# Autodesk Inventor assembly: Rat_Scanner_120_Ass
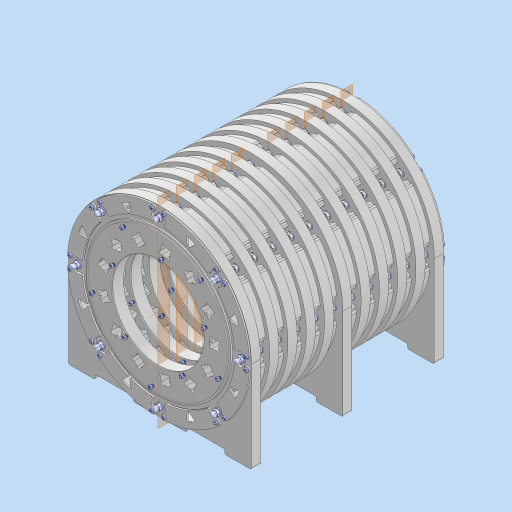
[picture p0: Inventor's stored thumbnail of the model, 512x512]
Saved by Autodesk Inventor 2024.2 (Build 282272000, 272)
## iProperties
Created: 2025-04-30
Part Number: Rat_Scanner_120_Ass
Document SubType Name: Assembly
Designer: 23661194
Author: 23661194
## Documents named in this file (14)
- C:\Users\23661194\OneDrive - Stellenbosch University\Master 2025 - Rat Scanner (120mm)\Rat_Scanner_120_V1\Rat_Scanner_120_Ass.iam
- C:\Users\23661194\OneDrive - Stellenbosch University\Master 2025 - Rat Scanner (120mm)\Rat_Scanner_120_V1\Ring_842_Sub.iam
- C:\Users\23661194\OneDrive - Stellenbosch University\Master 2025 - Rat Scanner (120mm)\Rat_Scanner_120_V1\Ring_945_Sub.iam
- C:\Users\23661194\OneDrive - Stellenbosch University\Master 2025 - Rat Scanner (120mm)\Rat_Scanner_120_V1\Ring_1050_Sub.iam
- C:\Users\23661194\OneDrive - Stellenbosch University\Master 2025 - Rat Scanner (120mm)\Rat_Scanner_120_V1\Ring_0_Sub.iam
- C:\Users\23661194\OneDrive - Stellenbosch University\Master 2025 - Rat Scanner (120mm)\Rat_Scanner_120_V1\Ring_1_Sub.iam
- C:\Users\23661194\OneDrive - Stellenbosch University\Master 2025 - Rat Scanner (120mm)\Rat_Scanner_120_V1\Ring_10_Sub.iam
- C:\Users\23661194\OneDrive - Stellenbosch University\Master 2025 - Rat Scanner (120mm)\Rat_Scanner_120_V1\Brass_Rod_M4.ipt
- C:\Users\23661194\OneDrive - Stellenbosch University\Master 2025 - Rat Scanner (120mm)\Rat_Scanner_120_V1\M4_Nylon_Washer.ipt
- C:\Users\23661194\OneDrive - Stellenbosch University\Master 2025 - Rat Scanner (120mm)\Rat_Scanner_120_V1\M4x3.2mm Hex Nut.ipt
- C:\Users\23661194\OneDrive - Stellenbosch University\Master 2025 - Rat Scanner (120mm)\Rat_Scanner_120_V1\M4 Dome Nut.ipt
- C:\Users\23661194\OneDrive - Stellenbosch University\Master 2025 - Rat Scanner (120mm)\Rat_Scanner_120_V1\Shim_Tray.ipt
- C:\Users\23661194\OneDrive - Stellenbosch University\Master 2025 - Rat Scanner (120mm)\Rat_Scanner_120_V1\Ring_10_Back_Sub.iam
- C:\Users\23661194\OneDrive - Stellenbosch University\Master 2025 - Rat Scanner (120mm)\Rat_Scanner_120_V1\M3x8.ipt
## Components (419 placed, 13 different names)
1. Ring_842_Sub:1 [sub-assembly] — Mate:1, Flush:1, Mate:2, Mate:3, Flush:2, Mate:4, Mate:5, Flush:3, Mate:7, Flush:4, Mate:10, Flush:5, Mate:12, Flush:6, Mate:15, Flush:7, Mate:17, Flush:8, Flush:10, Mate:51
2. Ring_945_Sub:1 [sub-assembly] — Mate:1, Flush:1, Mate:2, Mate:6, Mate:21, Flush:11
3. Ring_945_Sub:2 [sub-assembly] — Mate:3, Flush:2, Mate:4, Mate:8, Mate:39
4. Ring_1050_Sub:1 [sub-assembly] — Mate:5, Flush:3, Mate:6, Mate:9
5. Ring_1050_Sub:2 [sub-assembly] — Mate:7, Flush:4, Mate:8, Mate:11
6. Ring_0_Sub:1 [sub-assembly] — Mate:11, Mate:12, Flush:6, Mate:14
7. Ring_0_Sub:2 [sub-assembly] — Mate:9, Mate:10, Flush:5, Mate:16
8. Ring_1_Sub:1 [sub-assembly] — Mate:14, Mate:15, Flush:7, Mate:20
9. Ring_1_Sub:2 [sub-assembly] — Mate:16, Mate:17, Flush:8, Mate:38
10. Ring_10_Sub:2 [sub-assembly] — Mate:20, Mate:21, Flush:10, Mate:35, Mate:36, Mate:37, Mate:47, Mate:49, Mate:52
11. Ring_10_Back_Sub:1 [sub-assembly] — Mate:38, Mate:39, Flush:11, Mate:40, Mate:41, Mate:42, Mate:43, Mate:45, Flush:12, Mate:54
12. Shim_Tray:2 — Mate:40, Mate:41, Mate:42, Mate:44, Mate:46
13. M3x8:2 — Mate:45, Mate:46
14. M3x8:1 — Mate:43, Mate:44
15. Shim_Tray:3
16. M3x8:3
17. M3x8:4
18. Shim_Tray:4
19. M3x8:5
20. M3x8:6
21. Shim_Tray:5
22. M3x8:7
23. M3x8:8
24. Shim_Tray:6
25. M3x8:9
26. M3x8:10
27. Shim_Tray:7
28. M3x8:11
29. M3x8:12
30. Shim_Tray:8
31. M3x8:13
32. M3x8:14
33. Shim_Tray:9
34. M3x8:15
35. M3x8:16
36. Shim_Tray:1 — Mate:35, Mate:36, Mate:37, Mate:48, Mate:50
37. M3x8:17 — Mate:47, Mate:48
38. M3x8:18 — Mate:49, Mate:50
39. Shim_Tray:10
40. M3x8:19
41. M3x8:20
42. Shim_Tray:11
43. M3x8:21
44. M3x8:22
45. Shim_Tray:12
46. M3x8:23
47. M3x8:24
48. Shim_Tray:13
49. M3x8:25
50. M3x8:26
51. Shim_Tray:14
52. M3x8:27
53. M3x8:28
54. Shim_Tray:15
55. M3x8:29
56. M3x8:30
57. Shim_Tray:16
58. M3x8:31
59. M3x8:32
60. Brass_Rod_M4:1 — Mate:51, Flush:12
61. Brass_Rod_M4:2 — Mate:53, Mate:55, Mate:56, Mate:57, Mate:60, Mate:62
62. Brass_Rod_M4:3
63. Brass_Rod_M4:4
64. Brass_Rod_M4:5
65. Brass_Rod_M4:6
66. Brass_Rod_M4:7
67. Brass_Rod_M4:8
68. M4 Dome Nut:1 — Mate:56, Mate:59
69. M4 Dome Nut:2 — Mate:57, Mate:58
70. M4 Dome Nut:3
71. M4 Dome Nut:4
72. M4 Dome Nut:5
73. M4 Dome Nut:6
74. M4 Dome Nut:7
75. M4 Dome Nut:8
76. M4 Dome Nut:9
77. M4 Dome Nut:10
78. M4 Dome Nut:11
79. M4 Dome Nut:12
80. M4 Dome Nut:13
81. M4 Dome Nut:14
82. M4 Dome Nut:15
83. M4 Dome Nut:16
84. M4_Nylon_Washer:2 — Mate:52, Mate:53, Mate:59
85. M4_Nylon_Washer:3
86. M4_Nylon_Washer:4
87. M4_Nylon_Washer:5
88. M4_Nylon_Washer:6
89. M4_Nylon_Washer:7
90. M4_Nylon_Washer:8
91. M4_Nylon_Washer:9
92. M4_Nylon_Washer:10 — Mate:63
93. M4_Nylon_Washer:11
94. M4_Nylon_Washer:12
95. M4_Nylon_Washer:13
96. M4_Nylon_Washer:14
97. M4_Nylon_Washer:15
98. M4_Nylon_Washer:16
99. M4_Nylon_Washer:17
100. M4_Nylon_Washer:18
101. M4_Nylon_Washer:19
102. M4_Nylon_Washer:20
103. M4_Nylon_Washer:21
104. M4_Nylon_Washer:22
105. M4_Nylon_Washer:23
106. M4_Nylon_Washer:24
107. M4_Nylon_Washer:25
108. M4_Nylon_Washer:26
109. M4_Nylon_Washer:27
110. M4_Nylon_Washer:28
111. M4_Nylon_Washer:29
112. M4_Nylon_Washer:30
113. M4_Nylon_Washer:31
114. M4_Nylon_Washer:32
115. M4_Nylon_Washer:33
116. M4_Nylon_Washer:34
117. M4_Nylon_Washer:35
118. M4_Nylon_Washer:36
119. M4_Nylon_Washer:37
120. M4_Nylon_Washer:38
121. M4_Nylon_Washer:39
122. M4_Nylon_Washer:40
123. M4_Nylon_Washer:41
124. M4_Nylon_Washer:42
125. M4_Nylon_Washer:43
126. M4_Nylon_Washer:44
127. M4_Nylon_Washer:45
128. M4_Nylon_Washer:46
129. M4_Nylon_Washer:47
130. M4_Nylon_Washer:48
131. M4_Nylon_Washer:49
132. M4_Nylon_Washer:50
133. M4_Nylon_Washer:51
134. M4_Nylon_Washer:52
135. M4_Nylon_Washer:53
136. M4_Nylon_Washer:54
137. M4_Nylon_Washer:55
138. M4_Nylon_Washer:56
139. M4_Nylon_Washer:57
140. M4_Nylon_Washer:58
141. M4_Nylon_Washer:59
142. M4_Nylon_Washer:60
143. M4_Nylon_Washer:61
144. M4_Nylon_Washer:62
145. M4_Nylon_Washer:63
146. M4_Nylon_Washer:64
147. M4_Nylon_Washer:65
148. M4_Nylon_Washer:66
149. M4_Nylon_Washer:67
150. M4_Nylon_Washer:68
151. M4_Nylon_Washer:69
152. M4_Nylon_Washer:70
153. M4_Nylon_Washer:71
154. M4_Nylon_Washer:72
155. M4_Nylon_Washer:73
156. M4_Nylon_Washer:74
157. M4_Nylon_Washer:75
158. M4_Nylon_Washer:76
159. M4_Nylon_Washer:77
160. M4_Nylon_Washer:78
161. M4_Nylon_Washer:79
162. M4_Nylon_Washer:80
163. M4_Nylon_Washer:81
164. M4_Nylon_Washer:82
165. M4_Nylon_Washer:83
166. M4_Nylon_Washer:84
167. M4_Nylon_Washer:85
168. M4_Nylon_Washer:86
169. M4_Nylon_Washer:87
170. M4_Nylon_Washer:88
171. M4_Nylon_Washer:89
172. M4_Nylon_Washer:90 — Mate:54, Mate:55, Mate:58
173. M4_Nylon_Washer:91
174. M4_Nylon_Washer:92
175. M4_Nylon_Washer:93
176. M4_Nylon_Washer:94
177. M4_Nylon_Washer:95
178. M4_Nylon_Washer:96
179. M4_Nylon_Washer:97
180. M4_Nylon_Washer:98
181. M4_Nylon_Washer:99
182. M4_Nylon_Washer:100
183. M4_Nylon_Washer:101
184. M4_Nylon_Washer:102
185. M4_Nylon_Washer:103
186. M4_Nylon_Washer:104
187. M4_Nylon_Washer:105
188. M4_Nylon_Washer:106
189. M4_Nylon_Washer:107
190. M4_Nylon_Washer:108
191. M4_Nylon_Washer:109
192. M4_Nylon_Washer:110
193. M4_Nylon_Washer:111
194. M4_Nylon_Washer:112
195. M4_Nylon_Washer:113
196. M4_Nylon_Washer:114
197. M4_Nylon_Washer:115
198. M4_Nylon_Washer:116
199. M4_Nylon_Washer:117
200. M4_Nylon_Washer:118
201. M4_Nylon_Washer:119
202. M4_Nylon_Washer:120
203. M4_Nylon_Washer:121
204. M4_Nylon_Washer:122
205. M4_Nylon_Washer:123
206. M4_Nylon_Washer:124
207. M4_Nylon_Washer:125
208. M4_Nylon_Washer:126
209. M4_Nylon_Washer:127
210. M4_Nylon_Washer:128
211. M4_Nylon_Washer:129
212. M4_Nylon_Washer:130
213. M4_Nylon_Washer:131
214. M4_Nylon_Washer:132
215. M4_Nylon_Washer:133
216. M4_Nylon_Washer:134
217. M4_Nylon_Washer:135
218. M4_Nylon_Washer:136
219. M4_Nylon_Washer:137
220. M4_Nylon_Washer:138
221. M4_Nylon_Washer:139
222. M4_Nylon_Washer:140
223. M4_Nylon_Washer:141
224. M4_Nylon_Washer:142
225. M4_Nylon_Washer:143
226. M4_Nylon_Washer:144
227. M4_Nylon_Washer:145
228. M4_Nylon_Washer:146
229. M4_Nylon_Washer:147
230. M4_Nylon_Washer:148
231. M4_Nylon_Washer:149
232. M4_Nylon_Washer:150
233. M4_Nylon_Washer:151
234. M4_Nylon_Washer:152
235. M4_Nylon_Washer:153
236. M4_Nylon_Washer:154
237. M4_Nylon_Washer:155
238. M4_Nylon_Washer:156
239. M4_Nylon_Washer:157
240. M4_Nylon_Washer:158
241. M4_Nylon_Washer:159
242. M4_Nylon_Washer:160
243. M4_Nylon_Washer:161
244. M4_Nylon_Washer:162
245. M4_Nylon_Washer:163
246. M4_Nylon_Washer:164
247. M4_Nylon_Washer:165
248. M4_Nylon_Washer:166
249. M4_Nylon_Washer:167
250. M4_Nylon_Washer:168
251. M4_Nylon_Washer:169
252. M4_Nylon_Washer:170 — Mate:61
253. M4_Nylon_Washer:171
254. M4_Nylon_Washer:172
255. M4_Nylon_Washer:173
256. M4_Nylon_Washer:174
257. M4_Nylon_Washer:175
258. M4_Nylon_Washer:176
259. M4_Nylon_Washer:177
260. M4x3.2mm Hex Nut:2 — Mate:62, Mate:63
261. M4x3.2mm Hex Nut:1 — Mate:60, Mate:61
262. M4x3.2mm Hex Nut:3
263. M4x3.2mm Hex Nut:4
264. M4x3.2mm Hex Nut:5
265. M4x3.2mm Hex Nut:6
266. M4x3.2mm Hex Nut:7
267. M4x3.2mm Hex Nut:8
268. M4x3.2mm Hex Nut:9
269. M4x3.2mm Hex Nut:10
270. M4x3.2mm Hex Nut:11
271. M4x3.2mm Hex Nut:12
272. M4x3.2mm Hex Nut:13
273. M4x3.2mm Hex Nut:14
274. M4x3.2mm Hex Nut:15
275. M4x3.2mm Hex Nut:16
276. M4x3.2mm Hex Nut:17
277. M4x3.2mm Hex Nut:18
278. M4x3.2mm Hex Nut:19
279. M4x3.2mm Hex Nut:20
280. M4x3.2mm Hex Nut:21
281. M4x3.2mm Hex Nut:22
282. M4x3.2mm Hex Nut:23
283. M4x3.2mm Hex Nut:24
284. M4x3.2mm Hex Nut:25
285. M4x3.2mm Hex Nut:26
286. M4x3.2mm Hex Nut:27
287. M4x3.2mm Hex Nut:28
288. M4x3.2mm Hex Nut:29
289. M4x3.2mm Hex Nut:30
290. M4x3.2mm Hex Nut:31
291. M4x3.2mm Hex Nut:32
292. M4x3.2mm Hex Nut:33
293. M4x3.2mm Hex Nut:34
294. M4x3.2mm Hex Nut:35
295. M4x3.2mm Hex Nut:36
296. M4x3.2mm Hex Nut:37
297. M4x3.2mm Hex Nut:38
298. M4x3.2mm Hex Nut:39
299. M4x3.2mm Hex Nut:40
300. M4x3.2mm Hex Nut:41
301. M4x3.2mm Hex Nut:42
302. M4x3.2mm Hex Nut:43
303. M4x3.2mm Hex Nut:44
304. M4x3.2mm Hex Nut:45
305. M4x3.2mm Hex Nut:46
306. M4x3.2mm Hex Nut:47
307. M4x3.2mm Hex Nut:48
308. M4x3.2mm Hex Nut:49
309. M4x3.2mm Hex Nut:50
310. M4x3.2mm Hex Nut:51
311. M4x3.2mm Hex Nut:52
312. M4x3.2mm Hex Nut:53
313. M4x3.2mm Hex Nut:54
314. M4x3.2mm Hex Nut:55
315. M4x3.2mm Hex Nut:56
316. M4x3.2mm Hex Nut:57
317. M4x3.2mm Hex Nut:58
318. M4x3.2mm Hex Nut:59
319. M4x3.2mm Hex Nut:60
320. M4x3.2mm Hex Nut:61
321. M4x3.2mm Hex Nut:62
322. M4x3.2mm Hex Nut:63
323. M4x3.2mm Hex Nut:64
324. M4x3.2mm Hex Nut:65
325. M4x3.2mm Hex Nut:66
326. M4x3.2mm Hex Nut:67
327. M4x3.2mm Hex Nut:68
328. M4x3.2mm Hex Nut:69
329. M4x3.2mm Hex Nut:70
330. M4x3.2mm Hex Nut:71
331. M4x3.2mm Hex Nut:72
332. M4x3.2mm Hex Nut:73
333. M4x3.2mm Hex Nut:74
334. M4x3.2mm Hex Nut:75
335. M4x3.2mm Hex Nut:76
336. M4x3.2mm Hex Nut:77
337. M4x3.2mm Hex Nut:78
338. M4x3.2mm Hex Nut:79
339. M4x3.2mm Hex Nut:80
340. M4x3.2mm Hex Nut:81
341. M4x3.2mm Hex Nut:82
342. M4x3.2mm Hex Nut:83
343. M4x3.2mm Hex Nut:84
344. M4x3.2mm Hex Nut:85
345. M4x3.2mm Hex Nut:86
346. M4x3.2mm Hex Nut:87
347. M4x3.2mm Hex Nut:88
348. M4x3.2mm Hex Nut:89
349. M4x3.2mm Hex Nut:90
350. M4x3.2mm Hex Nut:91
351. M4x3.2mm Hex Nut:92
352. M4x3.2mm Hex Nut:93
353. M4x3.2mm Hex Nut:94
354. M4x3.2mm Hex Nut:95
355. M4x3.2mm Hex Nut:96
356. M4x3.2mm Hex Nut:97
357. M4x3.2mm Hex Nut:98
358. M4x3.2mm Hex Nut:99
359. M4x3.2mm Hex Nut:100
360. M4x3.2mm Hex Nut:101
361. M4x3.2mm Hex Nut:102
362. M4x3.2mm Hex Nut:103
363. M4x3.2mm Hex Nut:104
364. M4x3.2mm Hex Nut:105
365. M4x3.2mm Hex Nut:106
366. M4x3.2mm Hex Nut:107
367. M4x3.2mm Hex Nut:108
368. M4x3.2mm Hex Nut:109
369. M4x3.2mm Hex Nut:110
370. M4x3.2mm Hex Nut:111
371. M4x3.2mm Hex Nut:112
372. M4x3.2mm Hex Nut:113
373. M4x3.2mm Hex Nut:114
374. M4x3.2mm Hex Nut:115
375. M4x3.2mm Hex Nut:116
376. M4x3.2mm Hex Nut:117
377. M4x3.2mm Hex Nut:118
378. M4x3.2mm Hex Nut:119
379. M4x3.2mm Hex Nut:120
380. M4x3.2mm Hex Nut:121
381. M4x3.2mm Hex Nut:122
382. M4x3.2mm Hex Nut:123
383. M4x3.2mm Hex Nut:124
384. M4x3.2mm Hex Nut:125
385. M4x3.2mm Hex Nut:126
386. M4x3.2mm Hex Nut:127
387. M4x3.2mm Hex Nut:128
388. M4x3.2mm Hex Nut:129
389. M4x3.2mm Hex Nut:130
390. M4x3.2mm Hex Nut:131
391. M4x3.2mm Hex Nut:132
392. M4x3.2mm Hex Nut:133
393. M4x3.2mm Hex Nut:134
394. M4x3.2mm Hex Nut:135
395. M4x3.2mm Hex Nut:136
396. M4x3.2mm Hex Nut:137
397. M4x3.2mm Hex Nut:138
398. M4x3.2mm Hex Nut:139
399. M4x3.2mm Hex Nut:140
400. M4x3.2mm Hex Nut:141
401. M4x3.2mm Hex Nut:142
402. M4x3.2mm Hex Nut:143
403. M4x3.2mm Hex Nut:144
404. M4x3.2mm Hex Nut:145
405. M4x3.2mm Hex Nut:146
406. M4x3.2mm Hex Nut:147
407. M4x3.2mm Hex Nut:148
408. M4x3.2mm Hex Nut:149
409. M4x3.2mm Hex Nut:150
410. M4x3.2mm Hex Nut:151
411. M4x3.2mm Hex Nut:152
412. M4x3.2mm Hex Nut:153
413. M4x3.2mm Hex Nut:154
414. M4x3.2mm Hex Nut:155
415. M4x3.2mm Hex Nut:156
416. M4x3.2mm Hex Nut:157
417. M4x3.2mm Hex Nut:158
418. M4x3.2mm Hex Nut:159
419. M4x3.2mm Hex Nut:160
## Component patterns: (8 elements, first: Shim_Tray:2 + M3x8:2 + M3x8:1), (8 elements, first: Shim_Tray:1 + M3x8:17 + M3x8:18), (8 elements, first: Brass_Rod_M4:1), (11 elements), (11 elements), (8 elements, first: M4 Dome Nut:1 + M4 Dome Nut:2), (10 elements), (8 elements, first: M4_Nylon_Washer:2), Component Pattern 15:2 (8 elements), Component Pattern 15:3 (8 elements), Component Pattern 15:4 (8 elements), Component Pattern 15:5 (8 elements), Component Pattern 15:6 (8 elements), Component Pattern 15:7 (8 elements), Component Pattern 15:8 (8 elements), Component Pattern 15:9 (8 elements), Component Pattern 15:10 (8 elements), Component Pattern 15:11 (8 elements), (8 elements, first: M4_Nylon_Washer:90), Component Pattern 17:2 (8 elements), Component Pattern 17:3 (8 elements), Component Pattern 17:4 (8 elements), Component Pattern 17:5 (8 elements), Component Pattern 17:6 (8 elements), Component Pattern 17:7 (8 elements), Component Pattern 17:8 (8 elements), Component Pattern 17:9 (8 elements), Component Pattern 17:10 (8 elements), Component Pattern 17:11 (8 elements), (8 elements, first: M4x3.2mm Hex Nut:2 + M4x3.2mm Hex Nut:1), Component Pattern 20:2 (8 elements), Component Pattern 20:3 (8 elements), Component Pattern 20:4 (8 elements), Component Pattern 20:5 (8 elements), Component Pattern 20:6 (8 elements), Component Pattern 20:7 (8 elements), Component Pattern 20:8 (8 elements), Component Pattern 20:9 (8 elements), Component Pattern 20:10 (8 elements)
## Relationships (58: Mate 47, Flush 11)
- Mate:1: Ring_842_Sub:1 ↔ Ring_945_Sub:1
- Flush:1: Ring_842_Sub:1 ↔ Ring_945_Sub:1
- Mate:2 (12 mm): Ring_842_Sub:1 ↔ Ring_945_Sub:1
- Mate:3: Ring_842_Sub:1 ↔ Ring_945_Sub:2
- Flush:2: Ring_842_Sub:1 ↔ Ring_945_Sub:2
- Mate:4 (12 mm): Ring_842_Sub:1 ↔ Ring_945_Sub:2
- Mate:5: Ring_842_Sub:1 ↔ Ring_1050_Sub:1
- Flush:3: Ring_842_Sub:1 ↔ Ring_1050_Sub:1
- Mate:6 (12 mm): Ring_945_Sub:1 ↔ Ring_1050_Sub:1
- Mate:7: Ring_842_Sub:1 ↔ Ring_1050_Sub:2
- Flush:4: Ring_842_Sub:1 ↔ Ring_1050_Sub:2
- Mate:8 (12 mm): Ring_945_Sub:2 ↔ Ring_1050_Sub:2
- Mate:9 (12 mm): Ring_1050_Sub:1 ↔ Ring_0_Sub:2
- Mate:10: Ring_842_Sub:1 ↔ Ring_0_Sub:2
- Flush:5: Ring_842_Sub:1 ↔ Ring_0_Sub:2
- Mate:11 (12 mm): Ring_1050_Sub:2 ↔ Ring_0_Sub:1
- Mate:12: Ring_842_Sub:1 ↔ Ring_0_Sub:1
- Flush:6: Ring_842_Sub:1 ↔ Ring_0_Sub:1
- Mate:14 (12 mm): Ring_0_Sub:1 ↔ Ring_1_Sub:1
- Mate:15: Ring_842_Sub:1 ↔ Ring_1_Sub:1
- Flush:7: Ring_842_Sub:1 ↔ Ring_1_Sub:1
- Mate:16 (12 mm): Ring_0_Sub:2 ↔ Ring_1_Sub:2
- Mate:17: Ring_842_Sub:1 ↔ Ring_1_Sub:2
- Flush:8: Ring_842_Sub:1 ↔ Ring_1_Sub:2
- Mate:20 (12 mm): Ring_1_Sub:1 ↔ Ring_10_Sub:2
- Mate:21: Ring_945_Sub:1 ↔ Ring_10_Sub:2
- Flush:10: Ring_842_Sub:1 ↔ Ring_10_Sub:2
- Mate:35: Ring_10_Sub:2 ↔ Shim_Tray:1
- Mate:36: Ring_10_Sub:2 ↔ Shim_Tray:1
- Mate:37: Ring_10_Sub:2 ↔ Shim_Tray:1
- Mate:38 (12 mm): Ring_1_Sub:2 ↔ Ring_10_Back_Sub:1
- Mate:39: Ring_945_Sub:2 ↔ Ring_10_Back_Sub:1
- Flush:11: Ring_945_Sub:1 ↔ Ring_10_Back_Sub:1
- Mate:40: Ring_10_Back_Sub:1 ↔ Shim_Tray:2
- Mate:41: Ring_10_Back_Sub:1 ↔ Shim_Tray:2
- Mate:42: Ring_10_Back_Sub:1 ↔ Shim_Tray:2
- Mate:43: Ring_10_Back_Sub:1 ↔ M3x8:1
- Mate:44: Shim_Tray:2 ↔ M3x8:1
- Mate:45: Ring_10_Back_Sub:1 ↔ M3x8:2
- Mate:46: Shim_Tray:2 ↔ M3x8:2
- Mate:47: Ring_10_Sub:2 ↔ M3x8:17
- Mate:48: Shim_Tray:1 ↔ M3x8:17
- Mate:49: Ring_10_Sub:2 ↔ M3x8:18
- Mate:50: Shim_Tray:1 ↔ M3x8:18
- Mate:51: Ring_842_Sub:1 ↔ Brass_Rod_M4:1
- Flush:12 (-5 mm): Ring_10_Back_Sub:1 ↔ Brass_Rod_M4:1
- Mate:52: Ring_10_Sub:2 ↔ M4_Nylon_Washer:2
- Mate:53: Brass_Rod_M4:2 ↔ M4_Nylon_Washer:2
- Mate:54: Ring_10_Back_Sub:1 ↔ M4_Nylon_Washer:90
- Mate:55: Brass_Rod_M4:2 ↔ M4_Nylon_Washer:90
- Mate:56: Brass_Rod_M4:2 ↔ M4 Dome Nut:1
- Mate:57: Brass_Rod_M4:2 ↔ M4 Dome Nut:2
- Mate:58: M4 Dome Nut:2 ↔ M4_Nylon_Washer:90
- Mate:59: M4 Dome Nut:1 ↔ M4_Nylon_Washer:2
- Mate:60: Brass_Rod_M4:2 ↔ M4x3.2mm Hex Nut:1
- Mate:61: M4_Nylon_Washer:170 ↔ M4x3.2mm Hex Nut:1
- Mate:62: Brass_Rod_M4:2 ↔ M4x3.2mm Hex Nut:2
- Mate:63: M4_Nylon_Washer:10 ↔ M4x3.2mm Hex Nut:2
